# Autodesk Inventor assembly: Level 3 Assembly
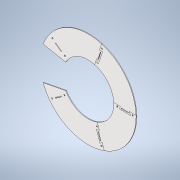
[picture p0: Inventor's stored thumbnail of the model, 180x180]
Saved by Autodesk Inventor 2020 (Build 240168000, 168)
## iProperties
Created: 2020-08-02
Part Number: Level 3 Assembly
Document SubType Name: Assembly
Designer: Dan Wikman
Author: Dan Wikman
## Documents named in this file (5)
- C:\Users\Dan Wikman\OneDrive\University Life\2020, Semester 1\METR4900 Honours Thesis\PROTOTYPE V2\Level 3 Assembly.iam
- C:\Users\Dan Wikman\OneDrive\University Life\2020, Semester 1\METR4900 Honours Thesis\PROTOTYPE V2\Level 3b - V2.ipt
- C:\Users\Dan Wikman\OneDrive\University Life\2020, Semester 1\METR4900 Honours Thesis\PROTOTYPE V2\Level 3c - V2.ipt
- C:\Users\Dan Wikman\OneDrive\University Life\2020, Semester 1\METR4900 Honours Thesis\PROTOTYPE V2\Level 3d - V2.ipt
- C:\Users\Dan Wikman\OneDrive\University Life\2020, Semester 1\METR4900 Honours Thesis\PROTOTYPE V2\Level 3a - V2.ipt
## Components (4 placed, 4 different names)
1. Level 3a - V2:1 — Flush:3, Mate:5, Mate:6
2. Level 3b - V2:1 — Flush:2, Mate:3, Mate:4, Flush:3, Mate:5, Mate:6
3. Level 3c - V2:1 — Flush:1, Mate:1, Mate:2, Flush:2, Mate:3, Mate:4
4. Level 3d - V2:1 — Flush:1, Mate:1, Mate:2
## Relationships (9: Mate 6, Flush 3)
- Flush:1: Level 3c - V2:1 ↔ Level 3d - V2:1
- Mate:1: Level 3c - V2:1 ↔ Level 3d - V2:1
- Mate:2: Level 3c - V2:1 ↔ Level 3d - V2:1
- Flush:2: Level 3b - V2:1 ↔ Level 3c - V2:1
- Mate:3: Level 3b - V2:1 ↔ Level 3c - V2:1
- Mate:4: Level 3b - V2:1 ↔ Level 3c - V2:1
- Flush:3: Level 3a - V2:1 ↔ Level 3b - V2:1
- Mate:5: Level 3a - V2:1 ↔ Level 3b - V2:1
- Mate:6: Level 3a - V2:1 ↔ Level 3b - V2:1
